# Autodesk Inventor assembly: Infinity
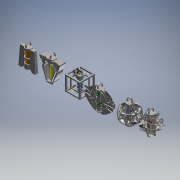
[picture p0: Inventor's stored thumbnail of the model, 180x180]
Saved by Autodesk Inventor 2019 (Build 230136000, 136)
## iProperties
Created: 2019-05-03
Part Number: Infinity
Document SubType Name: Assembly
Designer: Jorian Brusind
Author: Jorian Brusind
## Documents named in this file (7)
- C:\Users\Jorian Brusind\Documents\GitHub\PersonalProjects\Inventor Projects\Infinity\Infinity.iam
- C:\Users\Jorian Brusind\Documents\GitHub\PersonalProjects\Inventor Projects\Infinity\Time.iam
- C:\Users\Jorian Brusind\Documents\GitHub\PersonalProjects\Inventor Projects\Infinity\Space.iam
- C:\Users\Jorian Brusind\Documents\GitHub\PersonalProjects\Inventor Projects\Infinity\Power.iam
- C:\Users\Jorian Brusind\Documents\GitHub\PersonalProjects\Inventor Projects\Infinity\Mind.iam
- C:\Users\Jorian Brusind\Documents\GitHub\PersonalProjects\Inventor Projects\Infinity\Reality.iam
- C:\Users\Jorian Brusind\Documents\GitHub\PersonalProjects\Inventor Projects\Infinity\Soul.iam
## Components (6 placed, 6 different names)
1. Time:1 [sub-assembly] — Flush:1, Flush:4, Flush:8
2. Space:1 [sub-assembly] — Flush:1, Flush:4, Flush:6, Flush:7, Flush:9
3. Power:1 [sub-assembly] — Flush:8
4. Mind:1 [sub-assembly] — Flush:6, Flush:7
5. Reality:1 [sub-assembly] — Flush:9, Flush:10
6. Soul:1 [sub-assembly] — Flush:10
## Relationships (7: Flush 7)
- Flush:1: Time:1 ↔ Space:1
- Flush:4: Time:1 ↔ Space:1
- Flush:6: Space:1 ↔ Mind:1
- Flush:7: Space:1 ↔ Mind:1
- Flush:8: Time:1 ↔ Power:1
- Flush:9: Space:1 ↔ Reality:1
- Flush:10: Reality:1 ↔ Soul:1
